# Autodesk Inventor assembly: Head_camera_unit
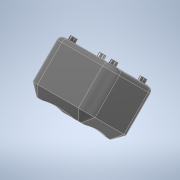
[picture p0: Inventor's stored thumbnail of the model, 180x180]
Saved by Autodesk Inventor 2022.3 (Build 263350000, 350)
## iProperties
Created: 2023-05-01
Part Number: Head_camera_unit
Document SubType Name: Assembly
Designer: Masato Kubotera
Author: Masato Kubotera
## Documents named in this file (4)
- C:\Users\Masato\Documents\Inventor\Inventor for CIT Brains\SUSTAINA-OP - mod\UpperBody\Head\Head_camera_unit.iam
- C:\Users\Masato\Documents\Inventor\Inventor for CIT Brains\SUSTAINA-OP - mod\UpperBody\Head\Head_camera_cover.iam
- C:\Users\Masato\Documents\Inventor\Inventor for CIT Brains\SUSTAINA-OP - mod\UpperBody\Head\Head_camera_unit_without_cover.iam
- C:\Users\Masato\Documents\Inventor\Inventor for CIT Brains\SUSTAINA-OP - mod\ReadyMade\Screw\UC-0308.ipt
## Components (6 placed, 3 different names)
1. Head_camera_cover:1 [sub-assembly] — Insert:1, Insert:2, Insert:3, Insert:4
2. Head_camera_unit_without_cover:1 [sub-assembly] — Insert:1, Insert:2, Insert:3, Insert:4, Insert:5, Insert:6, Insert:7, Insert:8, 角度:1, フラッシュ:1, メイト:1, メイト:2
3. UC-0308:1 — Insert:5
4. UC-0308:2 — Insert:6
5. UC-0308:3 — Insert:7
6. UC-0308:4 — Insert:8
## Relationships (12: Insert 8, Mate 2, Angle 1, Flush 1)
- Insert:1: Head_camera_cover:1 ↔ Head_camera_unit_without_cover:1
- Insert:2: Head_camera_cover:1 ↔ Head_camera_unit_without_cover:1
- Insert:3: Head_camera_cover:1 ↔ Head_camera_unit_without_cover:1
- Insert:4: Head_camera_cover:1 ↔ Head_camera_unit_without_cover:1
- Insert:5: Head_camera_unit_without_cover:1 ↔ UC-0308:1
- Insert:6: Head_camera_unit_without_cover:1 ↔ UC-0308:2
- Insert:7: Head_camera_unit_without_cover:1 ↔ UC-0308:3
- Insert:8: Head_camera_unit_without_cover:1 ↔ UC-0308:4
- 角度:1 [Angle] (45 deg): Head_camera_unit_without_cover:1
- フラッシュ:1 [Flush]: Head_camera_unit_without_cover:1
- メイト:1 [Mate]: Head_camera_unit_without_cover:1
- メイト:2 [Mate]: Head_camera_unit_without_cover:1
